# Autodesk Inventor assembly: Ring D Assembly
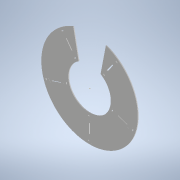
[picture p0: Inventor's stored thumbnail of the model, 180x180]
Saved by Autodesk Inventor 2020 (Build 240168000, 168)
## iProperties
Created: 2020-03-13
Part Number: Ring D Assembly
Document SubType Name: Assembly
Designer: Daniel Wikman
Author: Daniel Wikman
## Documents named in this file (5)
- C:\Users\Dan Wikman\OneDrive\University Life\2020, Semester 1\METR4900 Honours Thesis\Prototype CAD\Ring D Assembly.iam
- C:\Users\Dan Wikman\OneDrive\University Life\2020, Semester 1\METR4900 Honours Thesis\Prototype CAD\Ring D1.ipt
- C:\Users\Dan Wikman\OneDrive\University Life\2020, Semester 1\METR4900 Honours Thesis\Prototype CAD\Ring D2.ipt
- C:\Users\Dan Wikman\OneDrive\University Life\2020, Semester 1\METR4900 Honours Thesis\Prototype CAD\Ring D3.ipt
- C:\Users\Dan Wikman\OneDrive\University Life\2020, Semester 1\METR4900 Honours Thesis\Prototype CAD\Ring D4.ipt
## Components (4 placed, 4 different names)
1. Ring D1:1 — Flush:1, Mate:1, Mate:2
2. Ring D2:1 — Flush:1, Flush:2, Mate:1, Mate:2, Mate:3, Mate:4
3. Ring D3:1 — Flush:2, Flush:3, Mate:3, Mate:4, Mate:5, Mate:6
4. Ring D4:1 — Flush:3, Mate:5, Mate:6
## Relationships (9: Mate 6, Flush 3)
- Flush:1: Ring D1:1 ↔ Ring D2:1
- Flush:2: Ring D2:1 ↔ Ring D3:1
- Flush:3: Ring D3:1 ↔ Ring D4:1
- Mate:1: Ring D1:1 ↔ Ring D2:1
- Mate:2: Ring D1:1 ↔ Ring D2:1
- Mate:3: Ring D2:1 ↔ Ring D3:1
- Mate:4: Ring D2:1 ↔ Ring D3:1
- Mate:5: Ring D3:1 ↔ Ring D4:1
- Mate:6: Ring D3:1 ↔ Ring D4:1
